# Autodesk Inventor assembly: test1
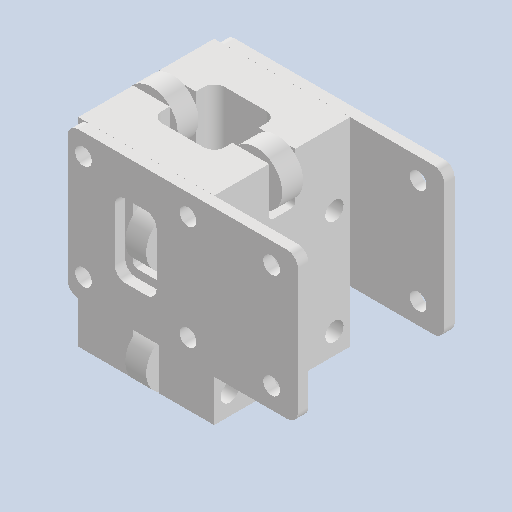
[picture p0: Inventor's stored thumbnail of the model, 512x512]
Saved by Autodesk Inventor 2025 (Build 290162000, 162)
## iProperties
Created: 2025-02-24
Part Number: test1
Document SubType Name: Assembly
Designer: Zhopa
Mass: 22.4539 g
Surface Area: 165.193 cm^2
Volume: 22.4539 cm^3
Density: 1 g/cm^3
Author: Zhopa
## Documents named in this file (4)
- C:\Users\onion\OneDrive - Kyushu University\共有用\工房共有ワンドライブ2024~2025用\ハード\NHK2025\Vova\elevator 3\subassemblies\carriage+holder_short.iam
- C:\Users\onion\OneDrive - Kyushu University\共有用\工房共有ワンドライブ2024~2025用\ハード\NHK2025\Vova\elevator 3\bearings\bearing 3-10x4.ipt
- C:\Users\onion\OneDrive - Kyushu University\共有用\工房共有ワンドライブ2024~2025用\ハード\NHK2025\Vova\elevator 3\3D printed\carriage_v1.ipt
- C:\Users\onion\OneDrive - Kyushu University\共有用\工房共有ワンドライブ2024~2025用\ハード\NHK2025\Vova\elevator 3\cnc\2mm_connect_short.ipt
## Components (11 placed, 3 different names)
1. bearing 3-10x4:1 — 挿入:1
2. carriage_v1:1 — 挿入:1, 挿入:2, 挿入:3, 挿入:4, 挿入:5, 挿入:6, 挿入:7, 挿入:8, 挿入:9, 挿入:10, 挿入:11, 挿入:12
3. bearing 3-10x4:2 — 挿入:6
4. bearing 3-10x4:3 — 挿入:7
5. bearing 3-10x4:7 — 挿入:8
6. bearing 3-10x4:10 — 挿入:4
7. bearing 3-10x4:11 — 挿入:2
8. bearing 3-10x4:12 — 挿入:3
9. bearing 3-10x4:13 — 挿入:5
10. 2mm_connect_short:1 — 挿入:9, 挿入:10
11. 2mm_connect_short:2 — 挿入:11, 挿入:12
## Relationships (12: Insert 12)
- 挿入:1 [Insert] (0.5 mm): bearing 3-10x4:1 ↔ carriage_v1:1
- 挿入:2 [Insert] (0.5 mm): carriage_v1:1 ↔ bearing 3-10x4:11
- 挿入:3 [Insert] (0.5 mm): carriage_v1:1 ↔ bearing 3-10x4:12
- 挿入:4 [Insert] (0.5 mm): carriage_v1:1 ↔ bearing 3-10x4:10
- 挿入:5 [Insert] (0.5 mm): carriage_v1:1 ↔ bearing 3-10x4:13
- 挿入:6 [Insert] (0.5 mm): carriage_v1:1 ↔ bearing 3-10x4:2
- 挿入:7 [Insert] (0.5 mm): carriage_v1:1 ↔ bearing 3-10x4:3
- 挿入:8 [Insert] (0.5 mm): carriage_v1:1 ↔ bearing 3-10x4:7
- 挿入:9 [Insert]: carriage_v1:1 ↔ 2mm_connect_short:1
- 挿入:10 [Insert]: carriage_v1:1 ↔ 2mm_connect_short:1
- 挿入:11 [Insert]: carriage_v1:1 ↔ 2mm_connect_short:2
- 挿入:12 [Insert]: carriage_v1:1 ↔ 2mm_connect_short:2
